# Autodesk Inventor assembly: Front Panel
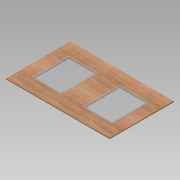
[picture p0: Inventor's stored thumbnail of the model, 180x180]
Saved by Autodesk Inventor 2015 (Build 190159000, 159)
## iProperties
Created: 2015-05-21
Part Number: Front Panel
Document SubType Name: Assembly
Designer: Joe Sheldon
Author: Joe Sheldon
## Documents named in this file (3)
- C:\Users\Joe Sheldon\Documents\PSU Stuff\PSU Clubs\Society of Physics Students\Cloud Chamber\Cloud Chamber CAD\Cart\Panelling\Front - Access\Front Panel.iam
- C:\Users\Joe Sheldon\Documents\PSU Stuff\PSU Clubs\Society of Physics Students\Cloud Chamber\Cloud Chamber CAD\Cart\Panelling\Front - Access\cart_woodpanel-front.ipt
- C:\Users\Joe Sheldon\Documents\PSU Stuff\PSU Clubs\Society of Physics Students\Cloud Chamber\Cloud Chamber CAD\Cart\Panelling\Front - Access\optix 8x10 window.ipt
## Components (3 placed, 2 different names)
1. cart_woodpanel-front:1 — Rigid:1, Rigid:2
2. optix 8x10 window:1 — Rigid:1
3. optix 8x10 window:2 — Rigid:2
## Relationships (2: WeldJoint 2)
- Rigid:1 [WeldJoint]: cart_woodpanel-front:1 ↔ optix 8x10 window:1
- Rigid:2 [WeldJoint]: cart_woodpanel-front:1 ↔ optix 8x10 window:2
